# Autodesk Inventor assembly: Ensa_carcasa
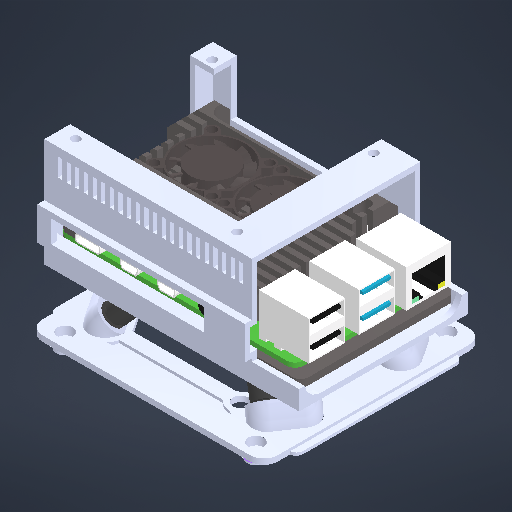
[picture p0: Inventor's stored thumbnail of the model, 512x512]
Saved by Autodesk Inventor 2026.2 (Build 302298000, 298)
## iProperties
Created: 2025-06-15
Part Number: Ensa_carcasa
Document SubType Name: Assembly
Designer: rodri
Mass: 131.895 g
Surface Area: 1100.1 cm^2
Volume: 93.6859 cm^3
Density: 1.40785 g/cm^3
Author: rodri
## Documents named in this file (5)
- D:\Documentos\inventor\Dron\Ensa_carcasa.iam
- D:\Documentos\inventor\Dron\1VibroNavio2bot_rev_A.ipt
- D:\Documentos\inventor\Dron\VibroNavio2top_rev_A.ipt
- D:\Documentos\inventor\Dron\antivibracion.ipt
- D:\Documentos\inventor\Dron\RPI4.ipt
## Components (11 placed, 4 different names)
1. 1VibroNavio2bot_rev_A:1 — Coincidencia:6, Coincidencia:7, Coincidencia:8, Coincidencia:9, Coincidencia:10, Coincidencia:11, Coincidencia:12, Coincidencia:13, Coincidencia:16, Coincidencia:17, Coincidencia:18
2. VibroNavio2top_rev_A:1 — Coincidencia:14, Coincidencia:15
3. antivibracion:1 — Coincidencia:7, Coincidencia:15
4. antivibracion:2 — Coincidencia:6
5. antivibracion:3 — Coincidencia:8
6. antivibracion:4 — Coincidencia:9
7. antivibracion:5 — Coincidencia:10
8. antivibracion:6 — Coincidencia:11
9. antivibracion:7 — Coincidencia:12
10. antivibracion:8 — Coincidencia:13, Coincidencia:14
11. RPI4:1 — Coincidencia:16, Coincidencia:17, Coincidencia:18
## Relationships (13: Mate 13)
- Coincidencia:6 [Mate]: 1VibroNavio2bot_rev_A:1 ↔ antivibracion:2
- Coincidencia:7 [Mate]: 1VibroNavio2bot_rev_A:1 ↔ antivibracion:1
- Coincidencia:8 [Mate]: 1VibroNavio2bot_rev_A:1 ↔ antivibracion:3
- Coincidencia:9 [Mate]: 1VibroNavio2bot_rev_A:1 ↔ antivibracion:4
- Coincidencia:10 [Mate]: 1VibroNavio2bot_rev_A:1 ↔ antivibracion:5
- Coincidencia:11 [Mate]: 1VibroNavio2bot_rev_A:1 ↔ antivibracion:6
- Coincidencia:12 [Mate]: 1VibroNavio2bot_rev_A:1 ↔ antivibracion:7
- Coincidencia:13 [Mate]: 1VibroNavio2bot_rev_A:1 ↔ antivibracion:8
- Coincidencia:14 [Mate]: VibroNavio2top_rev_A:1 ↔ antivibracion:8
- Coincidencia:15 [Mate]: VibroNavio2top_rev_A:1 ↔ antivibracion:1
- Coincidencia:16 [Mate]: 1VibroNavio2bot_rev_A:1 ↔ RPI4:1
- Coincidencia:17 [Mate]: 1VibroNavio2bot_rev_A:1 ↔ RPI4:1
- Coincidencia:18 [Mate]: 1VibroNavio2bot_rev_A:1 ↔ RPI4:1
